# Autodesk Inventor assembly: manual shifter_MIR
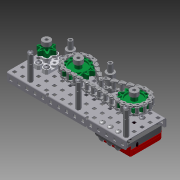
[picture p0: Inventor's stored thumbnail of the model, 180x180]
Saved by Autodesk Inventor 2014 SP1 (Build 180222100, 222)
## iProperties
Created: 2013-08-29
Part Number: manual shifter_MIR
Document SubType Name: Assembly
Designer: Ryan
Sending System: SolidWorks 2013
Last Author: Ryan
Author: Ryan
## Documents named in this file (21)
- C:\Users\Ryan\Desktop\pack and go\Workspaces\Workspace\toss up 1st A bot\inventor drive\manual shifter_MIR.iam
- C:\Users\Ryan\Desktop\pack and go\Workspaces\Workspace\lib\Aperture VEX CAD Library\Metal\C Channel\5 x 15.ipt
- C:\Users\Ryan\Desktop\pack and go\Workspaces\Workspace\lib\Aperture VEX CAD Library\Bearing Blocks\Bearing Block.ipt
- C:\Users\Ryan\Desktop\pack and go\Workspaces\Workspace\lib\Aperture VEX CAD Library\Hardware\8-32\8-32_.500.ipt
- C:\Users\Ryan\Desktop\pack and go\Workspaces\Workspace\lib\Super Sonic Sparks VEX CAD Library\Motors & Sensors\Optical Shaft (Quadrature) Encoder.iam
- C:\Users\Ryan\Desktop\pack and go\Workspaces\Workspace\lib\Aperture VEX CAD Library\Hardware\8-32\8-32_1.000.ipt
- C:\Users\Ryan\Desktop\pack and go\Workspaces\Workspace\lib\Aperture VEX CAD Library\Spacers\SPACER-0500-0125.ipt
- C:\Users\Ryan\Desktop\pack and go\Workspaces\Workspace\lib\Aperture VEX CAD Library\Hardware\Shaft Collar.ipt
- C:\Users\Ryan\Desktop\pack and go\Workspaces\Workspace\lib\Aperture VEX CAD Library\Sprockets\green\High Strength 12-Tooth Sprocket.ipt
- C:\Users\Ryan\Desktop\pack and go\Workspaces\Workspace\lib\Aperture VEX CAD Library\Spacers\spacer-0500-0250.ipt
- C:\Users\Ryan\Desktop\pack and go\Workspaces\Workspace\lib\Aperture VEX CAD Library\Spacers\spacer-0500-0500.ipt
- C:\Users\Ryan\Desktop\pack and go\Workspaces\Workspace\lib\Aperture VEX CAD Library\Sprockets\green\High Strength 6-Tooth Sprocket.ipt
- C:\Users\Ryan\Desktop\pack and go\Workspaces\Workspace\lib\Aperture VEX CAD Library\Hardware\8-32\8-32 nylock.ipt
- C:\Users\Ryan\Desktop\pack and go\Workspaces\Workspace\lib\Aperture VEX CAD Library\Standoffs\beam-0500.ipt
- C:\Users\Ryan\Desktop\pack and go\Workspaces\Workspace\lib\Aperture VEX CAD Library\Hardware\8-32\8-32 Nylock_MIR6.ipt
- C:\Users\Ryan\Desktop\pack and go\Workspaces\Workspace\toss up 1st A bot\inventor drive\manual shifter\Design Accelerator\V-Belt transmission1.iam
- C:\Users\Ryan\Desktop\pack and go\Workspaces\Workspace\lib\Aperture VEX CAD Library\Sprockets\HS Sprockets\High strength Chain Link.ipt
- C:\Users\Ryan\Desktop\pack and go\Workspaces\Workspace\toss up 1st A bot\inventor drive\manual shifter\Design Accelerator\V-Belt transmission2.iam
- C:\Users\Ryan\Desktop\pack and go\Workspaces\Workspace\lib\Aperture VEX CAD Library\Standoffs\BEAM-1000.ipt
- C:\Users\Ryan\Desktop\pack and go\Workspaces\Workspace\lib\Aperture VEX CAD Library\Hardware\8-32\8-32_.375.ipt
- C:\Users\Ryan\Desktop\pack and go\Workspaces\Workspace\lib\Aperture VEX CAD Library\Hardware\8-32\8-32_.875.ipt
## Components (122 placed, 19 different names)
1. 5 x 15:1 — Mate:63, Mate:68, Mate:69, Mate:76, Mate:54, Mate:2, Mate:1, Mate:7, Mate:8, Mate:9, Mate:42, Mate:47, Mate:15, Mate:23, Mate:67, Mate:66, Mate:62, Mate:44, Mate:43, Mate:28, Mate:26, Mate:24, Mate:18, Mate:17, Mate:16, Mate:14, Mate:13, Mate:12, Mate:4, Mate:3, Mate:74, Mate:73, Mate:72, Mate:94, Mate:95, Mate:99, Mate:98, Mate:103, Angle:1, Mate:115, Mate:120, Mate:114, Mate:113, Angle:2
2. Bearing Block:1 — Mate:63, Mate:65, Mate:64, Mate:81, Mate:55, Mate:67, Mate:66, Mate:62, Mate:106, Mate:107
3. 8-32_.500:1 — Mate:68, Mate:65, Mate:105
4. 8-32_.500:2 — Mate:69, Mate:64, Mate:104
5. Optical Shaft (Quadrature) Encoder:1 [sub-assembly] — Mate:81, Mate:79, Mate:77, Mate:71
6. SPACER-0500-0125:1 — Mate:55, Mate:54, Mate:57, Mate:56
7. Shaft Collar:1 — Mate:57, Mate:56, Mate:59, Mate:58
8. High Strength 12-Tooth Sprocket:1 — Mate:59, Mate:58, Mate:61, Mate:60
9. SPACER-0500-0250:1 — Mate:61, Mate:60, Mate:113
10. Bearing Block:2 — Mate:2, Mate:1, Mate:6, Mate:5, Mate:4, Mate:3, Mate:83, Mate:85
11. 8-32_.500:3 — Mate:7, Mate:6, Mate:82
12. 8-32_.500:4 — Mate:8, Mate:5, Mate:84
13. Bearing Block:3 — Mate:9, Mate:10, Mate:11, Mate:46, Mate:14, Mate:13, Mate:12, Mate:89, Mate:88
14. 8-32_.500:5 — Mate:10, Mate:86
15. 8-32_.500:6 — Mate:11, Mate:87
16. SPACER-0500-0250:2 — Mate:53, Mate:52, Mate:112
17. Shaft Collar:2 — Mate:49, Mate:48, Mate:51, Mate:50
18. SPACER-0500-0125:2 — Mate:49, Mate:48, Mate:47, Mate:46
19. High Strength 12-Tooth Sprocket:2 — Mate:53, Mate:52, Mate:51, Mate:50, Flush:1, Mate:114, Mate:115
20. Bearing Block:4 — Mate:15, Mate:39, Mate:38, Mate:37, Mate:20, Mate:18, Mate:17, Mate:16
21. 8-32_.500:7 — Mate:39, Mate:38, Mate:97, Mate:93
22. 8-32_.500:8 — Mate:37, Mate:20, Mate:90
23. 8-32_.500:9 — Mate:30, Mate:29, Mate:91
24. 8-32_.500:10 — Mate:27, Mate:25, Mate:96, Mate:92
25. Bearing Block:5 — Mate:30, Mate:29, Mate:27, Mate:25, Mate:23, Mate:32, Mate:31, Mate:28, Mate:26, Mate:24
26. SPACER-0500-0125:3 — Mate:32, Mate:31, Mate:34, Mate:33
27. High Strength 6-Tooth Sprocket:1 — Mate:34, Mate:33, Mate:36, Mate:35, Mate:108
28. SPACER-0500-0250:3 — Mate:36, Mate:35
29. 8-32 nylock:2 — Mate:83, Mate:82
30. 8-32 nylock:3 — Mate:85, Mate:84
31. 8-32 nylock:4 — Mate:89, Mate:86
32. 8-32 nylock:5 — Mate:88, Mate:87
33. 8-32 Nylock_MIR6:1 — Mate:94, Mate:91
34. 8-32 nylock:6 — Mate:95, Mate:90
35. 8-32 nylock:7 — Mate:99, Mate:97, Mate:93
36. 8-32 nylock:8 — Mate:98, Mate:96, Mate:92
37. 8-32 nylock:9 — Mate:106, Mate:105
38. 8-32 nylock:10 — Mate:107, Mate:104
39. V-Belt transmission:1 [sub-assembly]
40. High strength Chain Link:1 — Flush:1, Angle:1, Mate:108
41. High strength Chain Link:2
42. High strength Chain Link:3
43. High strength Chain Link:4
44. High strength Chain Link:5
45. High strength Chain Link:6
46. High strength Chain Link:7
47. High strength Chain Link:8
48. High strength Chain Link:9
49. High strength Chain Link:10
50. High strength Chain Link:11
51. High strength Chain Link:12
52. High strength Chain Link:13
53. High strength Chain Link:14
54. High strength Chain Link:15
55. High strength Chain Link:16
56. High strength Chain Link:17
57. High strength Chain Link:18
58. High strength Chain Link:19
59. High strength Chain Link:20
60. V-Belt transmission:2 [sub-assembly] — Mate:112, Mate:113, Mate:115
61. 8-32_1.000:1 — Mate:79, Mate:76, Mate:78, Mate:75
62. BEAM-0500:1 — Mate:75, Mate:74, Mate:73, Mate:72, Mate:71
63. 8-32 nylock:1 — Mate:78, Mate:77
64. 8-32_1.000:2
65. BEAM-0500:4
66. 8-32 nylock:11
67. 8-32_1.000:3
68. BEAM-0500:5
69. 8-32 nylock:12
70. BEAM-0500:2 — Mate:70, Mate:45
71. SPACER-0500-0500:2 — Mate:41, Mate:40, Mate:43, Mate:70, Mate:45
72. SPACER-0500-0500:1 — Mate:42, Mate:41, Mate:40, Mate:44, Mate:102
73. 8-32_.500:11 — Mate:103, Mate:102
74. BEAM-0500:6
75. SPACER-0500-0500:3
76. SPACER-0500-0500:4
77. 8-32_.500:12
78. BEAM-1000:1 — Mate:115, Mate:110, Flush:2, Mate:119, Mate:116
79. BEAM-0500:3 — Flush:2, Mate:119, Mate:116, Mate:118, Mate:117
80. 8-32_.875:1 — Mate:118, Mate:117
81. 8-32_.375:1 — Mate:120, Mate:114, Mate:113, Mate:110
82. BEAM-1000:2
83. BEAM-0500:7
84. 8-32_.875:2
85. 8-32_.375:2
86. BEAM-1000:3
87. BEAM-0500:8
88. 8-32_.875:3
89. 8-32_.375:3
90. High strength Chain Link:21 — Mate:114, Angle:2
91. High strength Chain Link:22
92. High strength Chain Link:23
93. High strength Chain Link:24
94. High strength Chain Link:25
95. High strength Chain Link:26
96. High strength Chain Link:27
97. High strength Chain Link:28
98. High strength Chain Link:29
99. High strength Chain Link:30
100. High strength Chain Link:31
101. High strength Chain Link:32
102. High strength Chain Link:33
103. High strength Chain Link:34
104. High strength Chain Link:35
105. High strength Chain Link:36
106. High strength Chain Link:37
107. High strength Chain Link:38
108. High strength Chain Link:39
109. High strength Chain Link:40
110. High strength Chain Link:41
111. High strength Chain Link:42
112. High strength Chain Link:43
113. High strength Chain Link:44
114. High strength Chain Link:45
115. High strength Chain Link:46
116. High strength Chain Link:47
117. High strength Chain Link:48
118. High strength Chain Link:49
119. High strength Chain Link:50
120. High strength Chain Link:51
121. High strength Chain Link:52
122. High strength Chain Link:53
## Component patterns: (3 elements, first: 8-32_1.000:1 + BEAM-0500:1 + 8-32 nylock:1), (2 elements, first: BEAM-0500:2 + SPACER-0500-0500:2 + SPACER-0500-0500:1 + 8-32_.500:11), (3 elements, first: BEAM-1000:1 + BEAM-0500:3 + 8-32_.875:1 + 8-32_.375:1), (33 elements, first: High strength Chain Link:21)
## Relationships (119: Mate 115, Flush 2, Angle 2)
- Mate:63: 5 x 15:1 ↔ Bearing Block:1
- Mate:68: 5 x 15:1 ↔ 8-32_.500:1
- Mate:65: Bearing Block:1 ↔ 8-32_.500:1
- Mate:69: 5 x 15:1 ↔ 8-32_.500:2
- Mate:64: Bearing Block:1 ↔ 8-32_.500:2
- Mate:81: Bearing Block:1 ↔ Optical Shaft (Quadrature) Encoder:1
- Mate:79 (2.25 mm): Optical Shaft (Quadrature) Encoder:1 ↔ 8-32_1.000:1
- Mate:76: 5 x 15:1 ↔ 8-32_1.000:1
- Mate:55: Bearing Block:1 ↔ SPACER-0500-0125:1
- Mate:54: 5 x 15:1 ↔ SPACER-0500-0125:1
- Mate:57: SPACER-0500-0125:1 ↔ Shaft Collar:1
- Mate:56: SPACER-0500-0125:1 ↔ Shaft Collar:1
- Mate:59: Shaft Collar:1 ↔ High Strength 12-Tooth Sprocket:1
- Mate:58: Shaft Collar:1 ↔ High Strength 12-Tooth Sprocket:1
- Mate:61: High Strength 12-Tooth Sprocket:1 ↔ SPACER-0500-0250:1
- Mate:60: High Strength 12-Tooth Sprocket:1 ↔ SPACER-0500-0250:1
- Mate:2: 5 x 15:1 ↔ Bearing Block:2
- Mate:1 (2.3114 mm): 5 x 15:1 ↔ Bearing Block:2
- Mate:7: 5 x 15:1 ↔ 8-32_.500:3
- Mate:6: Bearing Block:2 ↔ 8-32_.500:3
- Mate:8: 5 x 15:1 ↔ 8-32_.500:4
- Mate:5: Bearing Block:2 ↔ 8-32_.500:4
- Mate:9: 5 x 15:1 ↔ Bearing Block:3
- Mate:10: Bearing Block:3 ↔ 8-32_.500:5
- Mate:11: Bearing Block:3 ↔ 8-32_.500:6
- Mate:42: 5 x 15:1 ↔ SPACER-0500-0500:1
- Mate:41: SPACER-0500-0500:2 ↔ SPACER-0500-0500:1
- Mate:40: SPACER-0500-0500:2 ↔ SPACER-0500-0500:1
- Mate:49: Shaft Collar:2 ↔ SPACER-0500-0125:2
- Mate:48: Shaft Collar:2 ↔ SPACER-0500-0125:2
- Mate:47: 5 x 15:1 ↔ SPACER-0500-0125:2
- Mate:46: Bearing Block:3 ↔ SPACER-0500-0125:2
- Mate:53: SPACER-0500-0250:2 ↔ High Strength 12-Tooth Sprocket:2
- Mate:52: SPACER-0500-0250:2 ↔ High Strength 12-Tooth Sprocket:2
- Mate:51: Shaft Collar:2 ↔ High Strength 12-Tooth Sprocket:2
- Mate:50: Shaft Collar:2 ↔ High Strength 12-Tooth Sprocket:2
- Mate:15: 5 x 15:1 ↔ Bearing Block:4
- Mate:39: Bearing Block:4 ↔ 8-32_.500:7
- Mate:38: Bearing Block:4 ↔ 8-32_.500:7
- Mate:37: Bearing Block:4 ↔ 8-32_.500:8
- Mate:20: Bearing Block:4 ↔ 8-32_.500:8
- Mate:30: 8-32_.500:9 ↔ Bearing Block:5
- Mate:29: 8-32_.500:9 ↔ Bearing Block:5
- Mate:27: 8-32_.500:10 ↔ Bearing Block:5
- Mate:25: 8-32_.500:10 ↔ Bearing Block:5
- Mate:23: 5 x 15:1 ↔ Bearing Block:5
- Mate:32: Bearing Block:5 ↔ SPACER-0500-0125:3
- Mate:31: Bearing Block:5 ↔ SPACER-0500-0125:3
- Mate:34: SPACER-0500-0125:3 ↔ High Strength 6-Tooth Sprocket:1
- Mate:33: SPACER-0500-0125:3 ↔ High Strength 6-Tooth Sprocket:1
- Mate:36: High Strength 6-Tooth Sprocket:1 ↔ SPACER-0500-0250:3
- Mate:35: High Strength 6-Tooth Sprocket:1 ↔ SPACER-0500-0250:3
- Mate:78: 8-32_1.000:1 ↔ 8-32 nylock:1
- Mate:77: Optical Shaft (Quadrature) Encoder:1 ↔ 8-32 nylock:1
- Mate:67 (2.3114 mm): 5 x 15:1 ↔ Bearing Block:1
- Mate:66 (2.3114 mm): 5 x 15:1 ↔ Bearing Block:1
- Mate:62 (2.3114 mm): 5 x 15:1 ↔ Bearing Block:1
- Mate:44 (2.3114 mm): 5 x 15:1 ↔ SPACER-0500-0500:1
- Mate:43 (2.3114 mm): 5 x 15:1 ↔ SPACER-0500-0500:2
- Mate:28 (2.3114 mm): 5 x 15:1 ↔ Bearing Block:5
- Mate:26 (2.3114 mm): 5 x 15:1 ↔ Bearing Block:5
- Mate:24 (2.3114 mm): 5 x 15:1 ↔ Bearing Block:5
- Mate:18 (2.3114 mm): 5 x 15:1 ↔ Bearing Block:4
- Mate:17 (2.3114 mm): 5 x 15:1 ↔ Bearing Block:4
- Mate:16 (2.3114 mm): 5 x 15:1 ↔ Bearing Block:4
- Mate:14 (2.3114 mm): 5 x 15:1 ↔ Bearing Block:3
- Mate:13 (2.3114 mm): 5 x 15:1 ↔ Bearing Block:3
- Mate:12 (2.3114 mm): 5 x 15:1 ↔ Bearing Block:3
- Mate:4 (2.3114 mm): 5 x 15:1 ↔ Bearing Block:2
- Mate:3 (2.3114 mm): 5 x 15:1 ↔ Bearing Block:2
- Mate:75: 8-32_1.000:1 ↔ BEAM-0500:1
- Mate:74: 5 x 15:1 ↔ BEAM-0500:1
- Mate:73 (2.3114 mm): 5 x 15:1 ↔ BEAM-0500:1
- Mate:72 (2.3114 mm): 5 x 15:1 ↔ BEAM-0500:1
- Mate:71: Optical Shaft (Quadrature) Encoder:1 ↔ BEAM-0500:1
- Mate:70: BEAM-0500:2 ↔ SPACER-0500-0500:2
- Mate:45: BEAM-0500:2 ↔ SPACER-0500-0500:2
- Mate:83: Bearing Block:2 ↔ 8-32 nylock:2
- Mate:82: 8-32_.500:3 ↔ 8-32 nylock:2
- Mate:85: Bearing Block:2 ↔ 8-32 nylock:3
- Mate:84: 8-32_.500:4 ↔ 8-32 nylock:3
- Mate:89: Bearing Block:3 ↔ 8-32 nylock:4
- Mate:86: 8-32_.500:5 ↔ 8-32 nylock:4
- Mate:88: Bearing Block:3 ↔ 8-32 nylock:5
- Mate:87: 8-32_.500:6 ↔ 8-32 nylock:5
- Mate:94: 5 x 15:1 ↔ 8-32 Nylock_MIR6:1
- Mate:91: 8-32_.500:9 ↔ 8-32 Nylock_MIR6:1
- Mate:95: 5 x 15:1 ↔ 8-32 nylock:6
- Mate:90: 8-32_.500:8 ↔ 8-32 nylock:6
- Mate:99: 5 x 15:1 ↔ 8-32 nylock:7
- Mate:97: 8-32_.500:7 ↔ 8-32 nylock:7
- Mate:93: 8-32_.500:7 ↔ 8-32 nylock:7
- Mate:98: 5 x 15:1 ↔ 8-32 nylock:8
- Mate:96: 8-32_.500:10 ↔ 8-32 nylock:8
- Mate:92: 8-32_.500:10 ↔ 8-32 nylock:8
- Mate:103: 5 x 15:1 ↔ 8-32_.500:11
- Mate:102: SPACER-0500-0500:1 ↔ 8-32_.500:11
- Mate:106: Bearing Block:1 ↔ 8-32 nylock:9
- Mate:105: 8-32_.500:1 ↔ 8-32 nylock:9
- Mate:107: Bearing Block:1 ↔ 8-32 nylock:10
- Mate:104: 8-32_.500:2 ↔ 8-32 nylock:10
- Flush:1: High Strength 12-Tooth Sprocket:2 ↔ High strength Chain Link:1
- Angle:1 (348.5 deg): 5 x 15:1 ↔ High strength Chain Link:1
- Mate:108: High Strength 6-Tooth Sprocket:1 ↔ High strength Chain Link:1
- Mate:115: 5 x 15:1 ↔ BEAM-1000:1
- Mate:120 (2.3114 mm): 5 x 15:1 ↔ 8-32_.375:1
- Mate:114 (2.3114 mm): 5 x 15:1 ↔ 8-32_.375:1
- Mate:113: 5 x 15:1 ↔ 8-32_.375:1
- Mate:110: BEAM-1000:1 ↔ 8-32_.375:1
- Flush:2: BEAM-1000:1 ↔ BEAM-0500:3
- Mate:119: BEAM-1000:1 ↔ BEAM-0500:3
- Mate:116: BEAM-1000:1 ↔ BEAM-0500:3
- Mate:118 (1.1684 mm): BEAM-0500:3 ↔ 8-32_.875:1
- Mate:117: BEAM-0500:3 ↔ 8-32_.875:1
- Mate:112: SPACER-0500-0250:2 ↔ V-Belt transmission:2
- Mate:113: SPACER-0500-0250:1 ↔ V-Belt transmission:2
- Mate:114: High Strength 12-Tooth Sprocket:2 ↔ High strength Chain Link:21
- Angle:2 (32 deg): 5 x 15:1 ↔ High strength Chain Link:21
- Mate:115: High Strength 12-Tooth Sprocket:2 ↔ V-Belt transmission:2
